# Autodesk Inventor assembly: Baugruppe1
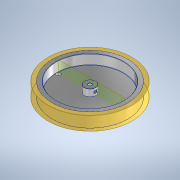
[picture p0: Inventor's stored thumbnail of the model, 180x180]
Saved by Autodesk Inventor 2022 (Build 260153000, 153)
## iProperties
Created: 2022-11-16
Part Number: Baugruppe1
Document SubType Name: Assembly
Designer: Friedrich Walmrath
Author: Friedrich Walmrath
## Documents named in this file (10)
- E:\Kartenzar70\Kartenzar70\CAD-Dateien\Abschusseinheit\simtest\Baugruppe1.iam
- E:\Kartenzar70\Kartenzar70\CAD-Dateien\Abschusseinheit\simtest\felge.ipt
- E:\Kartenzar70\Kartenzar70\CAD-Dateien\Abschusseinheit\simtest\reifen.ipt
- E:\Kartenzar70\Kartenzar70\CAD-Dateien\Abschusseinheit\simtest\nabe.ipt
- E:\Kartenzar70\Kartenzar70\CAD-Dateien\Abschusseinheit\simtest\Baugruppe1\AIP\FEA\e5l65niao.fins
- E:\Kartenzar70\Kartenzar70\CAD-Dateien\Abschusseinheit\simtest\Baugruppe1\AIP\FEA\e5l65niao.fsat
- E:\Kartenzar70\Kartenzar70\CAD-Dateien\Abschusseinheit\simtest\Baugruppe1\AIP\FEA\e5l65niao.ftes
- E:\Kartenzar70\Kartenzar70\CAD-Dateien\Abschusseinheit\simtest\Baugruppe1\AIP\FEA\e5l65niao.fwiz
- E:\Kartenzar70\Kartenzar70\CAD-Dateien\Abschusseinheit\simtest\Baugruppe1\AIP\FEA\e5l65nibk.fmsh
- E:\Kartenzar70\Kartenzar70\CAD-Dateien\Abschusseinheit\simtest\Baugruppe1\AIP\FEA\e5l65nibl.fres
## Components (3 placed, 3 different names)
1. felge:1 — Passend:1, Passend:2, Passend:3, Passend:4
2. reifen:1
3. nabe:1 — Passend:1, Passend:2, Passend:7, Passend:8
## Relationships (8: Mate 8)
- Passend:1 [Mate]: felge:1 ↔ nabe:1
- Passend:2 [Mate]: felge:1 ↔ nabe:1
- Passend:3 [Mate]: felge:1
- Passend:4 [Mate]: felge:1
- Passend:5 [Mate]
- Passend:6 [Mate]
- Passend:7 [Mate]: nabe:1
- Passend:8 [Mate]: nabe:1
## Named parameters: sa_0 = 2792.53, sa_1 = 0
note: some values were not read from the file. Shown as the stored number, unit unknown: "sa_0", "sa_1".
